# Autodesk Inventor assembly: box
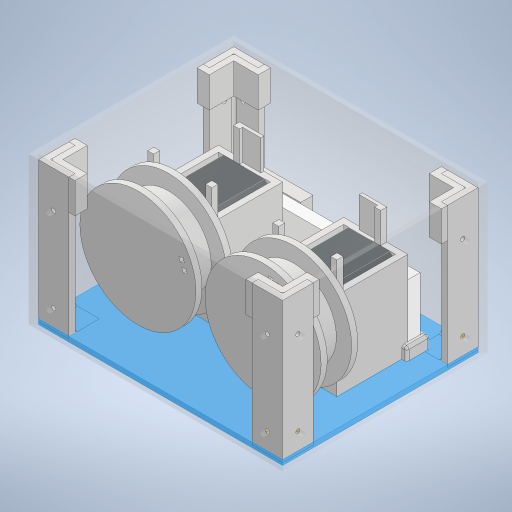
[picture p0: Inventor's stored thumbnail of the model, 512x512]
Saved by Autodesk Inventor 2023 (Build 270158000, 158)
## iProperties
Created: 2022-10-01
Part Number: box
Document SubType Name: Assembly
Designer: carso
Author: carso
## Documents named in this file (21)
- C:\Users\carso\OneDrive\Desktop\whiteboard\box.iam
- C:\Users\carso\OneDrive\Desktop\whiteboard\motor_mount.ipt
- C:\Users\carso\OneDrive\Desktop\whiteboard\stepper.ipt
- C:\Users\carso\OneDrive\Desktop\whiteboard\motor-shaft.ipt
- C:\Users\carso\OneDrive\Desktop\whiteboard\base.ipt
- C:\Users\carso\OneDrive\Desktop\whiteboard\breadboarde.ipt
- C:\Users\carso\OneDrive\Desktop\whiteboard\spool.ipt
- C:\Users\carso\OneDrive\Desktop\whiteboard\whiteboard-holder.ipt
- C:\Users\carso\OneDrive\Desktop\whiteboard\wall-joint.ipt
- C:\Users\carso\OneDrive\Desktop\whiteboard\m3_sizing_tests.ipt
- C:\Users\carso\OneDrive\Desktop\whiteboard\brick.ipt
- C:\Users\carso\OneDrive\Desktop\whiteboard\brick-clip.ipt
- C:\Users\carso\OneDrive\Desktop\whiteboard\brick-clip_MIR.ipt
- C:\Users\carso\OneDrive\Desktop\whiteboard\roof.ipt
- C:\Users\carso\OneDrive\Desktop\whiteboard\roof-joint.ipt
- C:\Users\carso\OneDrive\Desktop\whiteboard\roof-joint_MIR.ipt
- C:\Users\carso\OneDrive\Desktop\whiteboard\roof-joint_MIR1.ipt
- C:\Users\carso\OneDrive\Desktop\whiteboard\roof-joint_MIR_MIR.ipt
- C:\Users\carso\OneDrive\Desktop\whiteboard\wall-front.ipt
- C:\Users\carso\OneDrive\Desktop\whiteboard\wall-left.ipt
- C:\Users\carso\OneDrive\Desktop\whiteboard\fan.ipt
## Components (29 placed, 20 different names)
1. base:1 — Mate:24, Mate:25, Mate:26, Mate:27, Mate:29, Mate:40, Mate:41, Flush:9, Flush:10, Flush:11, Flush:12, Flush:13, Flush:14, Flush:15, Flush:16, Flush:17, Flush:18, Flush:19, Flush:20, Mate:46, Angle:3, Mate:69
2. breadboarde:1 — Mate:29, Mate:38, Flush:8, Mate:42
3. motor_mount:3 — Mate:14, Mate:25, Mate:27, Mate:31, Mate:48, Flush:21, Mate:49
4. stepper:3
5. motor-shaft:3 — Mate:15, Angle:1
6. spool:1 — Mate:14, Mate:15, Angle:1
7. motor_mount:4 — Mate:24, Mate:26, Mate:31, Mate:38, Mate:40, Flush:8, Mate:43, Mate:45
8. stepper:4
9. motor-shaft:4
10. spool:2
11. whiteboard-holder:1 — Mate:41, Mate:42, Mate:43
12. wall-joint:1 — Flush:9, Flush:10, Flush:11, Mate:59, Mate:63
13. m3_sizing_tests:1
14. brick:1 — Mate:45, Mate:47, Mate:48, Mate:50
15. wall-joint:2 — Flush:12, Flush:13, Flush:14, Flush:24, Mate:58, Mate:60, Symmetry:1, Mate:66
16. wall-joint:3 — Flush:15, Flush:16, Flush:17, Flush:25, Symmetry:1, Mate:62, Mate:65, Flush:70
17. wall-joint:4 — Flush:18, Flush:19, Flush:20, Mate:61, Mate:64
18. brick-clip:1 — Flush:21, Mate:49, Mate:50
19. brick-clip_MIR:1
20. roof:1 — Mate:52, Flush:24, Flush:25, Flush:26, Flush:27, Mate:54, Angle:4, Mate:55, Flush:28, Flush:29, Mate:56, Flush:30, Flush:31, Mate:57, Flush:32, Flush:33, Mate:58, Flush:34, Mate:67, Flush:69
21. roof-joint:1 — Mate:52, Flush:26, Flush:27
22. roof-joint_MIR:1 — Mate:55, Flush:28, Flush:29
23. roof-joint_MIR1:1 — Mate:57, Flush:32, Flush:33
24. roof-joint_MIR_MIR:1 — Mate:56, Flush:30, Flush:31
25. wall-front:1 — Mate:59, Mate:60, Mate:63, Mate:68
26. wall-front:2 — Mate:61, Mate:62, Mate:64
27. wall-left:1 — Mate:65, Flush:34, Mate:66
28. wall-left:2 — Mate:67, Flush:69, Mate:68
29. fan:1 — Mate:69, Flush:70
## Relationships (78: Mate 44, Flush 27, Angle 4, Insert 2, Symmetry 1)
- [Insert] (-22 mm): stepper:3 ↔ motor-shaft:3
- [Mate]: motor_mount:3 ↔ stepper:3
- [Mate]: motor_mount:3 ↔ stepper:3
- [Mate]: motor_mount:3 ↔ stepper:3
- Mate:14 (4 mm): motor_mount:3 ↔ spool:1
- Mate:15: motor-shaft:3 ↔ spool:1
- Angle:1 (-90 deg): motor-shaft:3 ↔ spool:1
- [Insert] (-22 mm): stepper:4 ↔ motor-shaft:4
- [Mate]: motor_mount:4 ↔ stepper:4
- [Mate]: motor_mount:4 ↔ stepper:4
- [Mate]: motor_mount:4 ↔ stepper:4
- [Mate] (4 mm): motor_mount:4 ↔ spool:2
- [Mate]: motor-shaft:4 ↔ spool:2
- [Angle] (-90 deg): motor-shaft:4 ↔ spool:2
- Mate:24: base:1 ↔ motor_mount:4
- Mate:25: base:1 ↔ motor_mount:3
- Mate:26: base:1 ↔ motor_mount:4
- Mate:27: base:1 ↔ motor_mount:3
- Mate:29: base:1 ↔ breadboarde:1
- Mate:31 (50 mm): motor_mount:3 ↔ motor_mount:4
- Mate:38: breadboarde:1 ↔ motor_mount:4
- Mate:40 (25 mm): base:1 ↔ motor_mount:4
- Flush:8: breadboarde:1 ↔ motor_mount:4
- Mate:41: base:1 ↔ whiteboard-holder:1
- Mate:42: breadboarde:1 ↔ whiteboard-holder:1
- Mate:43: motor_mount:4 ↔ whiteboard-holder:1
- Mate:45: motor_mount:4 ↔ brick:1
- Flush:9: base:1 ↔ wall-joint:1
- Flush:10: base:1 ↔ wall-joint:1
- Flush:11: base:1 ↔ wall-joint:1
- Flush:12: base:1 ↔ wall-joint:2
- Flush:13: base:1 ↔ wall-joint:2
- Flush:14: base:1 ↔ wall-joint:2
- Flush:15: base:1 ↔ wall-joint:3
- Flush:16: base:1 ↔ wall-joint:3
- Flush:17: base:1 ↔ wall-joint:3
- Flush:18: base:1 ↔ wall-joint:4
- Flush:19: base:1 ↔ wall-joint:4
- Flush:20: base:1 ↔ wall-joint:4
- Mate:46: base:1
- Angle:3 (90 deg): base:1
- Mate:47: brick:1
- Mate:48: motor_mount:3 ↔ brick:1
- Flush:21: motor_mount:3 ↔ brick-clip:1
- Mate:49: motor_mount:3 ↔ brick-clip:1
- Mate:50 (0.3 mm): brick:1 ↔ brick-clip:1
- Mate:52: roof:1 ↔ roof-joint:1
- Flush:24: wall-joint:2 ↔ roof:1
- Flush:25: wall-joint:3 ↔ roof:1
- Flush:26: roof:1 ↔ roof-joint:1
- Flush:27: roof:1 ↔ roof-joint:1
- Mate:54: roof:1
- Angle:4 (90 deg): roof:1
- Mate:55: roof:1 ↔ roof-joint_MIR:1
- Flush:28: roof:1 ↔ roof-joint_MIR:1
- Flush:29: roof:1 ↔ roof-joint_MIR:1
- Mate:56: roof:1 ↔ roof-joint_MIR_MIR:1
- Flush:30: roof:1 ↔ roof-joint_MIR_MIR:1
- Flush:31: roof:1 ↔ roof-joint_MIR_MIR:1
- Mate:57: roof:1 ↔ roof-joint_MIR1:1
- Flush:32: roof:1 ↔ roof-joint_MIR1:1
- Flush:33: roof:1 ↔ roof-joint_MIR1:1
- Mate:58: wall-joint:2 ↔ roof:1
- Mate:59: wall-joint:1 ↔ wall-front:1
- Mate:60: wall-joint:2 ↔ wall-front:1
- Symmetry:1: wall-joint:2 ↔ wall-joint:3
- Mate:61: wall-joint:4 ↔ wall-front:2
- Mate:62: wall-joint:3 ↔ wall-front:2
- Mate:63: wall-joint:1 ↔ wall-front:1
- Mate:64: wall-joint:4 ↔ wall-front:2
- Mate:65: wall-joint:3 ↔ wall-left:1
- Flush:34: roof:1 ↔ wall-left:1
- Mate:66: wall-joint:2 ↔ wall-left:1
- Mate:67: roof:1 ↔ wall-left:2
- Flush:69: roof:1 ↔ wall-left:2
- Mate:68: wall-front:1 ↔ wall-left:2
- Mate:69: base:1 ↔ fan:1
- Flush:70: wall-joint:3 ↔ fan:1
## Named parameters: d14_d7_d0 = -22 mm, d15_d8 = 0 mm, d16_d9 = 0 mm, d17_d10 = 0 mm, d34_d27 = 4 mm, d35_d28 = 0 mm, d36_d29 = -90 deg, d37_d14_d7_d0 = -22 mm, d38_d15_d8 = 0 mm, d39_d16_d9 = 0 mm, d40_d17_d10 = 0 mm
